# Autodesk Inventor assembly: ASY SLM FDS way1_1600
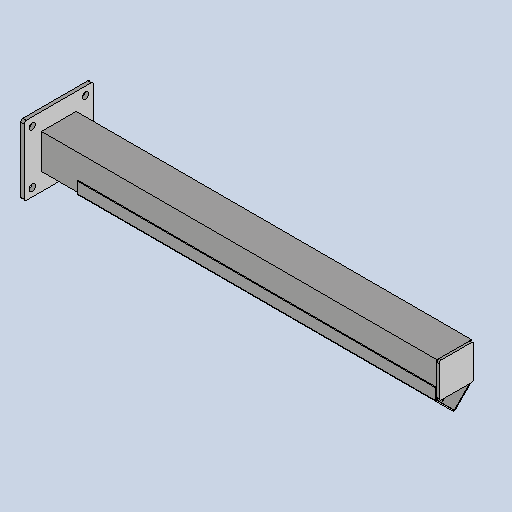
[picture p0: Inventor's stored thumbnail of the model, 512x512]
Saved by Autodesk Inventor 2025.3 (Build 293356030, 356C)
## iProperties
Created: 2025-07-02
Part Number: ASY SLM FDS way1_1600
Document SubType Name: Assembly
Designer: admin
Author: user
## Documents named in this file (5)
- C:\Users\admin\Documents\Inventor\NDA-Nyyda\ASY PNS FDS way1_1600.iam
- C:\Users\admin\Documents\Inventor\NDA-Nyyda\PNS 1661 FDS 1000 way tube 1.ipt
- C:\Users\admin\Documents\Inventor\NDA-Nyyda\PNS 1666 FDS 1000 CUP 1.ipt
- C:\Users\admin\Documents\Inventor\NDA-Nyyda\SLM 1425 FDS Way FLANGE.ipt
- C:\Users\admin\Documents\Inventor\NDA-Nyyda\NDA-512 roof 2.ipt
## Components (4 placed, 4 different names)
1. PNS 1661 FDS 1000 way tube 1.ipt:1 — Rigid:13, Rigid:14, Rigid:15
2. PNS 1666 FDS 1000 CUP 1.ipt:1 — Rigid:13
3. NDA-512 roof 2:1 — Rigid:15
4. SLM 1425 FDS Way FLANGE:1 — Rigid:14
## Relationships (3: WeldJoint 3)
- Rigid:13 [WeldJoint]: PNS 1661 FDS 1000 way tube 1.ipt:1 ↔ PNS 1666 FDS 1000 CUP 1.ipt:1
- Rigid:14 [WeldJoint]: PNS 1661 FDS 1000 way tube 1.ipt:1 ↔ SLM 1425 FDS Way FLANGE:1
- Rigid:15 [WeldJoint]: PNS 1661 FDS 1000 way tube 1.ipt:1 ↔ NDA-512 roof 2:1
